# Autodesk Inventor assembly: 01-03-02 Zange rechts
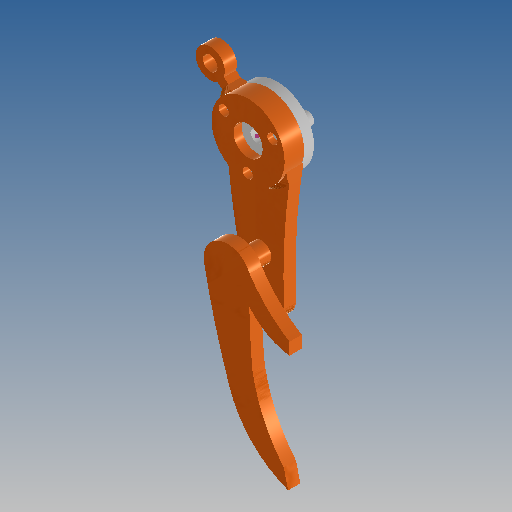
[picture p0: Inventor's stored thumbnail of the model, 512x512]
Saved by Autodesk Inventor 2026.2 (Build 302298000, 298)
## iProperties
Created: 2026-01-31
Part Number: 01-03-02 Zange rechts
Document SubType Name: Assembly
Designer: Schally
Author: Schally
## Documents named in this file (5)
- E:\06 Carologistics\02 Zeichnungen Greifer System\Gripper Version 2 speziell deutsche Meisterschaft\01-03-02 Zange rechts.iam
- E:\06 Carologistics\02 Zeichnungen Greifer System\Gripper Version 2 speziell deutsche Meisterschaft\01-03-02-01 Zeichnung Zange rechts.ipt
- E:\06 Carologistics\02 Zeichnungen Greifer System\Gripper Version 2 speziell deutsche Meisterschaft\01-03-02-02 Zeichnung Zange rechts oben.ipt
- E:\06 Carologistics\02 Zeichnungen Greifer System\Gripper Version 2 speziell deutsche Meisterschaft\01-03-01-03 Schraube kl.ipt
- E:\06 Carologistics\02 Zeichnungen Greifer System\Gripper Version 2 speziell deutsche Meisterschaft\01-03-01-04 Kugellager Tarik.ipt
## Components (6 placed, 4 different names)
1. 01-03-02-01 Zeichnung Zange rechts:1 — Einfügen:4, Einfügen:5, Einfügen:6
2. 01-03-02-02 Zeichnung Zange rechts oben:1 — Einfügen:1, Einfügen:2, Einfügen:3, Einfügen:4, Einfügen:5
3. 01-03-01-03 Schraube kl:1 — Einfügen:1
4. 01-03-01-03 Schraube kl:2 — Einfügen:3
5. 01-03-01-03 Schraube kl:3 — Einfügen:2
6. 01-03-01-04 Kugellager Tarik:1 — Einfügen:6
## Relationships (6: Insert 6)
- Einfügen:1 [Insert]: 01-03-02-02 Zeichnung Zange rechts oben:1 ↔ 01-03-01-03 Schraube kl:1
- Einfügen:2 [Insert]: 01-03-02-02 Zeichnung Zange rechts oben:1 ↔ 01-03-01-03 Schraube kl:3
- Einfügen:3 [Insert]: 01-03-02-02 Zeichnung Zange rechts oben:1 ↔ 01-03-01-03 Schraube kl:2
- Einfügen:4 [Insert]: 01-03-02-01 Zeichnung Zange rechts:1 ↔ 01-03-02-02 Zeichnung Zange rechts oben:1
- Einfügen:5 [Insert]: 01-03-02-01 Zeichnung Zange rechts:1 ↔ 01-03-02-02 Zeichnung Zange rechts oben:1
- Einfügen:6 [Insert]: 01-03-02-01 Zeichnung Zange rechts:1 ↔ 01-03-01-04 Kugellager Tarik:1
